# Autodesk Inventor assembly: modularRICH
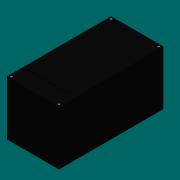
[picture p0: Inventor's stored thumbnail of the model, 180x180]
Saved by Autodesk Inventor 2016 SP1 (Build 200210100, 210)
## iProperties
Created: 2015-10-13
Part Number: modularRICH
Document SubType Name: Assembly
Designer: Sawaiz
Author: Sawaiz
## Documents named in this file (7)
- C:\Users\sawai\OneDrive\projects\modularRICH\modularRICH.iam
- C:\Users\sawai\OneDrive\projects\modularRICH\frame\frame.iam
- C:\Users\sawai\OneDrive\projects\modularRICH\fresnelLens.ipt
- C:\Users\sawai\OneDrive\projects\modularRICH\mirror\mirrorHolder.iam
- C:\Users\sawai\OneDrive\projects\modularRICH\aerogel.ipt
- C:\Users\sawai\OneDrive\projects\modularRICH\detector\fourPmtDetector.iam
- C:\Users\sawai\OneDrive\projects\modularRICH\modularRICH.xlsx
## Components (5 placed, 5 different names)
1. frame:1 [sub-assembly] — Mate:2, Mate:3, Mate:4, Mate:6, Mate:7
2. mirrorHolder:1 [sub-assembly] — Mate:1, Flush:1, Flush:2, Mate:2, Mate:3, Mate:4, Mate:5
3. fresnelLens:1 — Mate:1, Flush:1, Flush:2
4. aerogel:1
5. fourPmtDetector:1 [sub-assembly] — Mate:5, Mate:6, Mate:7
## Relationships (9: Mate 7, Flush 2)
- Mate:1: mirrorHolder:1 ↔ fresnelLens:1
- Flush:1: mirrorHolder:1 ↔ fresnelLens:1
- Flush:2: mirrorHolder:1 ↔ fresnelLens:1
- Mate:2: frame:1 ↔ mirrorHolder:1
- Mate:3: frame:1 ↔ mirrorHolder:1
- Mate:4: frame:1 ↔ mirrorHolder:1
- Mate:5: mirrorHolder:1 ↔ fourPmtDetector:1
- Mate:6: frame:1 ↔ fourPmtDetector:1
- Mate:7: frame:1 ↔ fourPmtDetector:1
## Named parameters: acrylicThickness = 6.35 mm, aerogelThickness = 30 mm, height = 127 mm, width = 127 mm, depth = 273.05 mm, mirrorAngle = 5 deg, detectorWidth = 52 mm, detectorHeight = 52 mm, mirrorThickness = 3.175 mm, fresnelThickness = 0.1 mm, grooveDensity = 100, focalLength = 76.2 mm, ior = 1.49, centerThickness = 1.524 mm, fresnelAngle = 90 deg, fresnelEffectiveDiameter = 152.4 mm, mirrorSuppourtWidth = 38.1 mm, backGrooveBit = 4.8006 mm, sensorHolderWidth = 88.9 mm, sensorHolderSesnorHeight = 53.975 mm, sensorHolderSensorWidth = 53.975 mm, sensorHolderHeight = 88.9 mm, sensorHolderSensorHeight = 53.975 mm, sensorHolderORingGroove = 3.175 mm, sensorHolderORing = 3.175 mm, sensorHolderFlushORingID = 304.8 mm, sensorHolderFlushORing = 3.175 mm, oRingWidth = 1.5875 mm, sensorHolderORingID = 203.2 mm, frontBackORingID = 419.1 mm, topBottomHorizontalMirrorGroove = 12.7 mm, backMirrorGroove = 6.35 mm, mirrorGroove = 19.05 mm, compressionPercent = 40, fresnelChamfer = 6.35 mm, mirrorGrooveFillet = 6.35 mm, mirrorGrooveDrill = 6.35 mm, mirrorGrooveMill = 3.175 mm, fresnelMirrorChamfer = 6.35 mm, detectorOpeningHeight = 76.2 mm, detectorOpeningWidth = 76.2 mm, sensorHolderDepth = 19.05 mm, aerogelHeight = 110 mm, aerogelWidth = 110 mm, frameAcrylicThickness = 9.525 mm, internalAcrylicThicnkess = 6.35 mm, internalAcrylicThickness = 6.35 mm, aerogelClearence = 3.175 mm, backplanePCBWidth = 76.2 mm, backplanePCBHeight = 76.2 mm, backplaneHoleOffsett = 6.35 mm, backplanePostionOffsett = 12.7 mm, moduleSlotClearence = 0.79375 mm, testMountWidth = 300 mm, testMountHeight = 300 mm, testMountLength = 500 mm
